# Autodesk Inventor assembly: guide
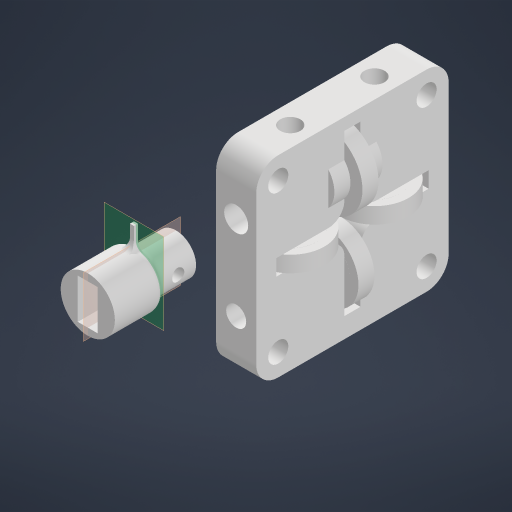
[picture p0: Inventor's stored thumbnail of the model, 512x512]
Saved by Autodesk Inventor 2024 (Build 280153000, 153)
## iProperties
Created: 2026-03-27
Part Number: guide
Document SubType Name: Assembly
Designer: schar
Author: schar
## Documents named in this file (7)
- C:\Users\schar\Desktop\FloatingFace\models\guide.iam
- C:\Users\schar\Desktop\FloatingFace\models\guidance_block.ipt
- C:\Users\schar\Desktop\FloatingFace\models\guide_bearing_assembly.iam
- C:\Users\schar\Desktop\FloatingFace\models\695_bearing.ipt
- C:\Users\schar\Desktop\FloatingFace\models\counter_wheel.ipt
- C:\Users\schar\Desktop\FloatingFace\models\counter_shaft.ipt
- C:\Users\schar\Desktop\FloatingFace\models\measurments_axis_holder.ipt
## Components (9 placed, 6 different names)
1. guidance_block:1 — Mate:1, Mate:2, Mate:3, Mate:4, Mate:7, Mate:8, Flush:1, Angle:1, Flush:3, Mate:9, Mate:10, Mate:11, Mate:12, Mate:13
2. guide_bearing_assembly:1 [sub-assembly] — Mate:1, Mate:2
3. guide_bearing_assembly:2 [sub-assembly] — Mate:7, Mate:8
4. guide_bearing_assembly:3 [sub-assembly] — Mate:3, Mate:4
5. 695_bearing:1 — Mate:9, Mate:10, Flush:5
6. 695_bearing:2 — Mate:11, Mate:12, Flush:4
7. counter_wheel:1 — Flush:4
8. counter_shaft:1 — Mate:13, Flush:5, Mate:14, Mate:15, Flush:6, Angle:2
9. measurments_axis_holder:1 — Mate:14, Mate:15, Angle:2
## Relationships (21: Mate 13, Flush 6, Angle 2)
- Mate:1: guidance_block:1 ↔ guide_bearing_assembly:1
- Mate:2: guidance_block:1 ↔ guide_bearing_assembly:1
- Mate:3: guidance_block:1 ↔ guide_bearing_assembly:3
- Mate:4: guidance_block:1 ↔ guide_bearing_assembly:3
- Mate:7: guidance_block:1 ↔ guide_bearing_assembly:2
- Mate:8: guidance_block:1 ↔ guide_bearing_assembly:2
- Flush:1 (-24 mm): guidance_block:1
- Angle:1 (0 deg): guidance_block:1
- Flush:2 (-1.172 mm)
- Flush:3: guidance_block:1
- Mate:9: guidance_block:1 ↔ 695_bearing:1
- Mate:10: guidance_block:1 ↔ 695_bearing:1
- Mate:11: guidance_block:1 ↔ 695_bearing:2
- Mate:12: guidance_block:1 ↔ 695_bearing:2
- Flush:4: 695_bearing:2 ↔ counter_wheel:1
- Mate:13: guidance_block:1 ↔ counter_shaft:1
- Flush:5: 695_bearing:1 ↔ counter_shaft:1
- Mate:14: counter_shaft:1 ↔ measurments_axis_holder:1
- Mate:15: counter_shaft:1 ↔ measurments_axis_holder:1
- Flush:6: counter_shaft:1
- Angle:2 (0 deg): counter_shaft:1 ↔ measurments_axis_holder:1
